# Autodesk Inventor assembly: vexFrisbeeShooter10
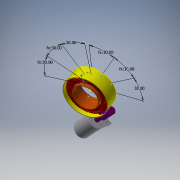
[picture p0: Inventor's stored thumbnail of the model, 180x180]
Saved by Autodesk Inventor 2016 SP1 (Build 200210100, 210)
## iProperties
Created: 2015-11-02
Part Number: vexFrisbeeShooter10
Document SubType Name: Assembly
Designer: steele
Author: steele
## Documents named in this file (9)
- C:\snobotics\CAD-Development\robSteele\FRC 2013 Ultimate Ascent\vexFrisbeeShooter10.iam
- C:\snobotics\CAD-Development\robSteele\FRC 2013 Ultimate Ascent\vexFrisbeeShooter10\Design Accelerator\Worm Gears1.iam
- C:\snobotics\CAD-MfgResources\VexRobotics\Motors\Vex Mini Cim 217-3371.ipt
- C:\snobotics\CAD-MfgResources\Andy-Mark\MotorMounts\AM 2488 CIM bracket.ipt
- C:\snobotics\CAD-Development\robSteele\FRC 2013 Ultimate Ascent\LexanBasePlate.ipt
- C:\snobotics\CAD-Development\robSteele\FRC 2013 Ultimate Ascent\vexInnerFrisbeeHopper.ipt
- C:\snobotics\CAD-Development\robSteele\FRC 2013 Ultimate Ascent\vexOuterFrisbeeHopper.ipt
- C:\snobotics\CAD-Development\robSteele\FRC 2013 Ultimate Ascent\wormGearSupport.ipt
- C:\snobotics\CAD-Development\robSteele\FRC 2013 Ultimate Ascent\vexCamPost10.ipt
## Components (8 placed, 8 different names)
1. Worm Gears:1 [sub-assembly] — Insert:1, Insert:3, Insert:6, Insert:7
2. Vex Mini Cim 217-3371:1 — Insert:1, Insert:2
3. AM 2488 CIM bracket:1 — Insert:2
4. LexanBasePlate:1 — Insert:3, Insert:4, Insert:5
5. vexInnerFrisbeeHopper:1 — Insert:4
6. vexOuterFrisbeeHopper:1 — Insert:5
7. wormGearSupport:1 — Insert:6
8. vexCamPost10:1 — Insert:7
## Relationships (7: Insert 7)
- Insert:1: Worm Gears:1 ↔ Vex Mini Cim 217-3371:1
- Insert:2: Vex Mini Cim 217-3371:1 ↔ AM 2488 CIM bracket:1
- Insert:3 (33.3502 mm): Worm Gears:1 ↔ LexanBasePlate:1
- Insert:4: LexanBasePlate:1 ↔ vexInnerFrisbeeHopper:1
- Insert:5: LexanBasePlate:1 ↔ vexOuterFrisbeeHopper:1
- Insert:6: Worm Gears:1 ↔ wormGearSupport:1
- Insert:7: Worm Gears:1 ↔ vexCamPost10:1
